# Autodesk Inventor assembly: power_distribution
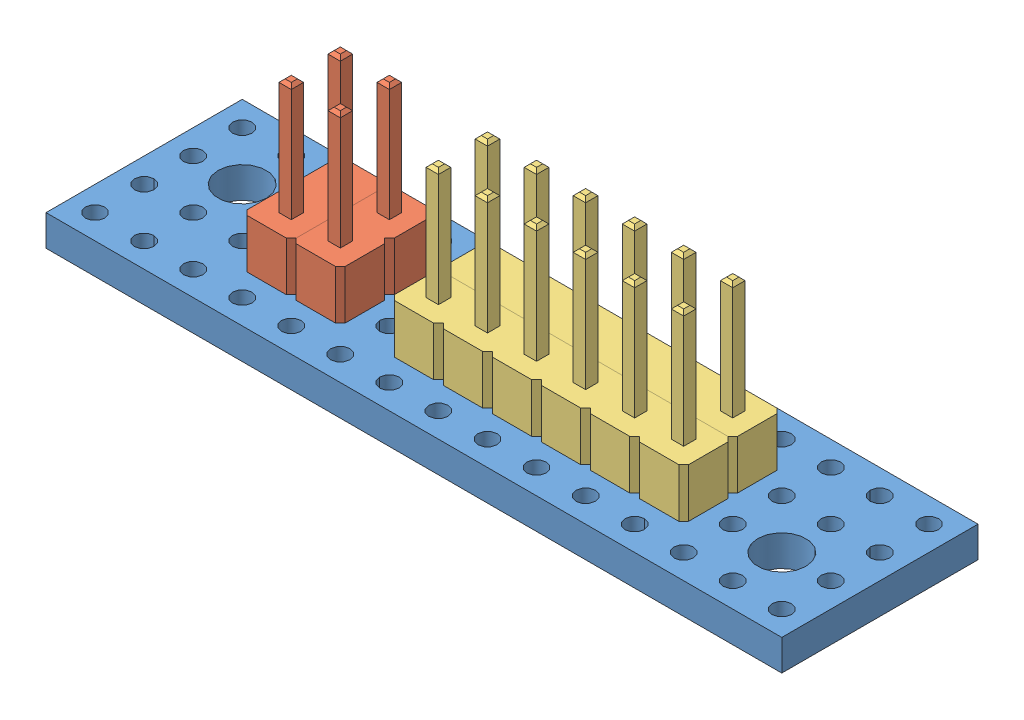
[picture p0: shaded view drawn from the shape stored in the file]
Saved by Autodesk Inventor 2021 (Build 250183000, 183)
## iProperties
Created: 2021-01-22
Part Number: power_distribution
Document SubType Name: Assembly
Designer: User
Author: User
## Documents named in this file (4)
- D:\SynologyDrive\tcodev\tco-cad\common\power_distribution\power_distribution.iam
- D:\SynologyDrive\tcodev\tco-cad\common\power_distribution\Board.ipt
- D:\SynologyDrive\tcodev\tco-cad\common\kicad_packages_3d\PinHeader_1x02_P2.54mm_Vertical.ipt
- D:\SynologyDrive\tcodev\tco-cad\common\kicad_packages_3d\PinHeader_1x06_P2.54mm_Vertical.ipt
## Components (5 placed, 3 different names)
1. Board:1 — Mate:1, Mate:2, Mate:3, Mate:4, Rigid:1, Rigid:2, Rigid:3, Rigid:4
2. PinHeader_1x02_P2.54mm_Vertical:1 — Mate:1, Rigid:1
3. PinHeader_1x02_P2.54mm_Vertical:2 — Mate:2, Rigid:2
4. PinHeader_1x06_P2.54mm_Vertical:1 — Mate:3, Rigid:4
5. PinHeader_1x06_P2.54mm_Vertical:2 — Mate:4, Rigid:3
## Relationships (8: Mate 4, WeldJoint 4)
- Mate:1: Board:1 ↔ PinHeader_1x02_P2.54mm_Vertical:1
- Mate:2: Board:1 ↔ PinHeader_1x02_P2.54mm_Vertical:2
- Mate:3: Board:1 ↔ PinHeader_1x06_P2.54mm_Vertical:1
- Mate:4: Board:1 ↔ PinHeader_1x06_P2.54mm_Vertical:2
- Rigid:1 [WeldJoint] (-3 mm): Board:1 ↔ PinHeader_1x02_P2.54mm_Vertical:1
- Rigid:2 [WeldJoint] (-3 mm): Board:1 ↔ PinHeader_1x02_P2.54mm_Vertical:2
- Rigid:3 [WeldJoint] (-3 mm): Board:1 ↔ PinHeader_1x06_P2.54mm_Vertical:2
- Rigid:4 [WeldJoint] (-3 mm): Board:1 ↔ PinHeader_1x06_P2.54mm_Vertical:1
